# Autodesk Inventor assembly: Base + Motor and Gear Apparatus
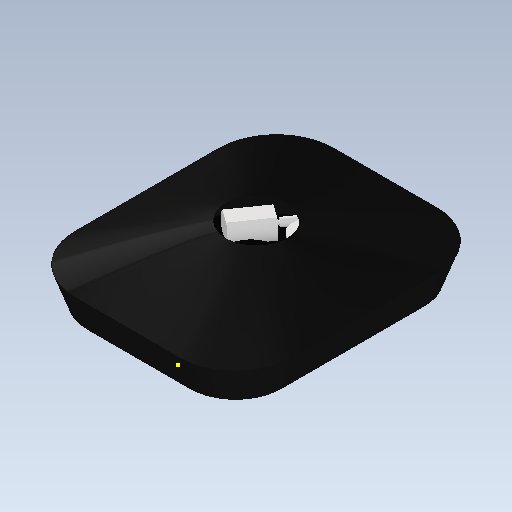
[picture p0: Inventor's stored thumbnail of the model, 512x512]
Saved by Autodesk Inventor 2021 (Build 250183000, 183)
## iProperties
Created: 2020-12-03
Part Number: Base + Motor and Gear Apparatus
Document SubType Name: Assembly
Designer: leoulgezu18
Author: leoulgezu18
## Documents named in this file (4)
- C:\Users\leoul\Desktop\Kinect 3D Modeling-20201204T005715Z-001\Kinect 3D Modeling\Sub-assemblies\Base + Motor and Gear Apparatus.iam
- C:\Users\leoul\Desktop\Kinect 3D Modeling-20201204T005715Z-001\Kinect 3D Modeling\Parts\Base Bottom.ipt
- C:\Users\leoul\Desktop\Kinect 3D Modeling-20201204T005715Z-001\Kinect 3D Modeling\Parts\base top.ipt
- C:\Users\leoul\Desktop\Kinect 3D Modeling-20201204T005715Z-001\Kinect 3D Modeling\Parts\Motor and gear apparatus\Gear base almost finished.iam
## Components (3 placed, 3 different names)
1. Base Bottom:1 — Mate:1, Insert:1, Angle:1, Mate:2
2. base top:1 — Angle:1, Mate:2
3. Gear base almost finished:1 [sub-assembly] — Mate:1, Insert:1
## Relationships (4: Mate 2, Insert 1, Angle 1)
- Mate:1: Base Bottom:1 ↔ Gear base almost finished:1
- Insert:1: Base Bottom:1 ↔ Gear base almost finished:1
- Angle:1 (180 deg): Base Bottom:1 ↔ base top:1
- Mate:2: Base Bottom:1 ↔ base top:1
